# Autodesk Inventor assembly: 00_031_THORAX_R1
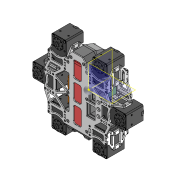
[picture p0: Inventor's stored thumbnail of the model, 180x180]
Saved by Autodesk Inventor 2021.2 (Build 252289000, 289)
## iProperties
Created: 2018-08-06
Part Number: 00_031_THORAX_R1
Material: 一般
Document SubType Name: Assembly
Designer: student
Mass: 676.028 g
Surface Area: 2162.31 cm^2
Volume: 512.52 cm^3
Density: 1.31903 g/cm^3
Author: student
## Documents named in this file (11)
- C:\Workspace\HaptHexa\Hardware\Inventor\00_031_THORAX_R1.iam
- C:\Workspace\HaptHexa\Hardware\Inventor\00_044_THORAX_YAW_R1.iam
- C:\Workspace\HaptHexa\Hardware\Inventor\20_042_BATTERY_R1.ipt
- C:\Workspace\HaptHexa\Hardware\Inventor\20_032_U2D2_TRANSCEIVER_R1.ipt
- C:\Workspace\HaptHexa\Hardware\Inventor\16_039_BOTTOM_CHASSIS_R1.ipt
- C:\Workspace\HaptHexa\Hardware\Inventor\16_041_TOP_CHASSIS_RIGHT_R1.ipt
- C:\Workspace\HaptHexa\Hardware\Inventor\15_034_BODY_FRAME_R2.ipt
- C:\Workspace\HaptHexa\Hardware\Inventor\16_035_BATTERY_HOLDER_BACK_R1.ipt
- C:\Workspace\HaptHexa\Hardware\Inventor\00_033_BATTERY_LIB_R1.iam
- C:\Workspace\HaptHexa\Hardware\Inventor\16_040_TOP_CHASSIS_LEFT_R1.ipt
- C:\Workspace\HaptHexa\Hardware\Inventor\21_043_PROCESSOR_PCB_R1.ipt
## Components (15 placed, 10 different names)
1. 15_034_BODY_FRAME_R2:1 — フラッシュ:1, フラッシュ:2, フラッシュ:3, メイト:46, メイト:47, メイト:48, メイト:49, Flush:54, Mate:67, Mate:68, Mate:69
2. 20_042_BATTERY_R1:1 — Mate:65, Mate:66, Flush:54
3. 20_032_U2D2_TRANSCEIVER_R1:1 — メイト:46, メイト:48
4. 16_039_BOTTOM_CHASSIS_R1:1 — メイト:4, メイト:5, Mate:17, Mate:18, Mate:23, Mate:24, メイト:26, メイト:27, フラッシュ:51, Flush:52, Flush:53, メイト:49, メイト:52, メイト:53, メイト:54, Flush:63, Mate:56, Mate:57, Flush:64, Mate:59, Mate:60, Mate:66
5. 00_033_BATTERY_LIB_R1:1 [sub-assembly] — Mate:64, Mate:70
6. 16_041_TOP_CHASSIS_RIGHT_R1:1 — メイト:42, Mate:43, Flush:6
7. 16_040_TOP_CHASSIS_LEFT_R1:1 — Flush:62, Mate:62, Mate:63
8. 21_043_PROCESSOR_PCB_R1:1 — メイト:47, フラッシュ:49, フラッシュ:50
9. 16_035_BATTERY_HOLDER_BACK_R1:1 — Mate:67, Mate:68, Mate:69, Mate:70
10. 00_044_THORAX_YAW_R1:4 [sub-assembly] — メイト:52, メイト:53, メイト:54, Mate:62, Mate:63
11. 00_044_THORAX_YAW_R1:5 [sub-assembly] — Mate:56, Mate:57, Flush:62, Flush:64
12. 00_044_THORAX_YAW_R1:6 [sub-assembly] — Mate:59, Mate:60, Flush:63
13. 00_044_THORAX_YAW_R1:1 [sub-assembly] — メイト:26, メイト:27, フラッシュ:51
14. 00_044_THORAX_YAW_R1:2 [sub-assembly] — Mate:23, Mate:24, メイト:42, Mate:43, Flush:52
15. 00_044_THORAX_YAW_R1:3 [sub-assembly] — Mate:17, Mate:18, Flush:53, Flush:6
## Relationships (43: Mate 30, Flush 13)
- メイト:4 [Mate]: 16_039_BOTTOM_CHASSIS_R1:1
- メイト:5 [Mate]: 16_039_BOTTOM_CHASSIS_R1:1
- フラッシュ:1 [Flush]: 15_034_BODY_FRAME_R2:1
- フラッシュ:2 [Flush] (-13 mm): 15_034_BODY_FRAME_R2:1
- フラッシュ:3 [Flush]: 15_034_BODY_FRAME_R2:1
- Mate:17: 16_039_BOTTOM_CHASSIS_R1:1 ↔ 00_044_THORAX_YAW_R1:3
- Mate:18: 16_039_BOTTOM_CHASSIS_R1:1 ↔ 00_044_THORAX_YAW_R1:3
- Mate:23: 16_039_BOTTOM_CHASSIS_R1:1 ↔ 00_044_THORAX_YAW_R1:2
- Mate:24: 16_039_BOTTOM_CHASSIS_R1:1 ↔ 00_044_THORAX_YAW_R1:2
- メイト:26 [Mate]: 16_039_BOTTOM_CHASSIS_R1:1 ↔ 00_044_THORAX_YAW_R1:1
- メイト:27 [Mate]: 16_039_BOTTOM_CHASSIS_R1:1 ↔ 00_044_THORAX_YAW_R1:1
- メイト:42 [Mate]: 16_041_TOP_CHASSIS_RIGHT_R1:1 ↔ 00_044_THORAX_YAW_R1:2
- Mate:43: 16_041_TOP_CHASSIS_RIGHT_R1:1 ↔ 00_044_THORAX_YAW_R1:2
- Flush:6: 16_041_TOP_CHASSIS_RIGHT_R1:1 ↔ 00_044_THORAX_YAW_R1:3
- メイト:46 [Mate] (3 mm): 15_034_BODY_FRAME_R2:1 ↔ 20_032_U2D2_TRANSCEIVER_R1:1
- メイト:47 [Mate]: 15_034_BODY_FRAME_R2:1 ↔ 21_043_PROCESSOR_PCB_R1:1
- フラッシュ:49 [Flush]: 21_043_PROCESSOR_PCB_R1:1
- フラッシュ:50 [Flush]: 21_043_PROCESSOR_PCB_R1:1
- メイト:48 [Mate]: 15_034_BODY_FRAME_R2:1 ↔ 20_032_U2D2_TRANSCEIVER_R1:1
- フラッシュ:51 [Flush]: 16_039_BOTTOM_CHASSIS_R1:1 ↔ 00_044_THORAX_YAW_R1:1
- Flush:52: 16_039_BOTTOM_CHASSIS_R1:1 ↔ 00_044_THORAX_YAW_R1:2
- Flush:53: 16_039_BOTTOM_CHASSIS_R1:1 ↔ 00_044_THORAX_YAW_R1:3
- メイト:49 [Mate]: 15_034_BODY_FRAME_R2:1 ↔ 16_039_BOTTOM_CHASSIS_R1:1
- メイト:52 [Mate]: 16_039_BOTTOM_CHASSIS_R1:1 ↔ 00_044_THORAX_YAW_R1:4
- メイト:53 [Mate]: 16_039_BOTTOM_CHASSIS_R1:1 ↔ 00_044_THORAX_YAW_R1:4
- メイト:54 [Mate]: 16_039_BOTTOM_CHASSIS_R1:1 ↔ 00_044_THORAX_YAW_R1:4
- Flush:63: 16_039_BOTTOM_CHASSIS_R1:1 ↔ 00_044_THORAX_YAW_R1:6
- Mate:56: 16_039_BOTTOM_CHASSIS_R1:1 ↔ 00_044_THORAX_YAW_R1:5
- Mate:57: 16_039_BOTTOM_CHASSIS_R1:1 ↔ 00_044_THORAX_YAW_R1:5
- Flush:64: 16_039_BOTTOM_CHASSIS_R1:1 ↔ 00_044_THORAX_YAW_R1:5
- Mate:59: 16_039_BOTTOM_CHASSIS_R1:1 ↔ 00_044_THORAX_YAW_R1:6
- Mate:60: 16_039_BOTTOM_CHASSIS_R1:1 ↔ 00_044_THORAX_YAW_R1:6
- Flush:62: 16_040_TOP_CHASSIS_LEFT_R1:1 ↔ 00_044_THORAX_YAW_R1:5
- Mate:62: 16_040_TOP_CHASSIS_LEFT_R1:1 ↔ 00_044_THORAX_YAW_R1:4
- Mate:63: 16_040_TOP_CHASSIS_LEFT_R1:1 ↔ 00_044_THORAX_YAW_R1:4
- Mate:64: 00_033_BATTERY_LIB_R1:1
- Mate:65: 20_042_BATTERY_R1:1
- Mate:66: 20_042_BATTERY_R1:1 ↔ 16_039_BOTTOM_CHASSIS_R1:1
- Flush:54: 15_034_BODY_FRAME_R2:1 ↔ 20_042_BATTERY_R1:1
- Mate:67: 15_034_BODY_FRAME_R2:1 ↔ 16_035_BATTERY_HOLDER_BACK_R1:1
- Mate:68: 15_034_BODY_FRAME_R2:1 ↔ 16_035_BATTERY_HOLDER_BACK_R1:1
- Mate:69: 15_034_BODY_FRAME_R2:1 ↔ 16_035_BATTERY_HOLDER_BACK_R1:1
- Mate:70: 00_033_BATTERY_LIB_R1:1 ↔ 16_035_BATTERY_HOLDER_BACK_R1:1
